# Autodesk Inventor assembly: Assembly10
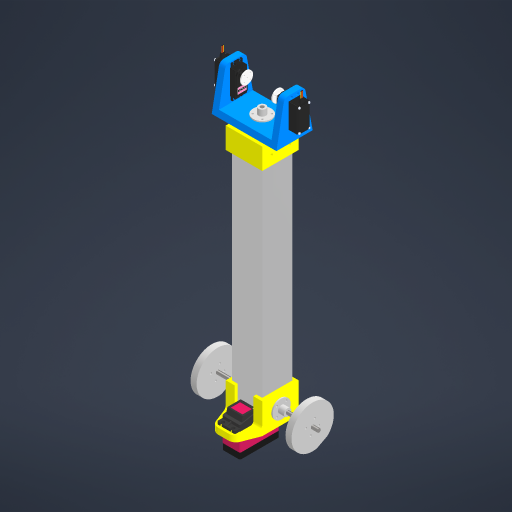
[picture p0: Inventor's stored thumbnail of the model, 512x512]
Saved by Autodesk Inventor 2023 (Build 270158000, 158)
## iProperties
Created: 2023-08-13
Part Number: Assembly10
Document SubType Name: Assembly
Designer: Abhinav
Author: Abhinav
## Documents named in this file (11)
- C:\Users\Abhinav\Desktop\GRID\ARM 3\Hand\00_Hand.iam
- C:\Users\Abhinav\Desktop\3D Library\60 kg cm Servo.ipt
- C:\Users\Abhinav\Desktop\GRID\ARM 3\Hand\Hand-Link.ipt
- C:\Users\Abhinav\Desktop\GRID\ARM 3\Hand\Servo-house.ipt
- C:\Users\Abhinav\Desktop\GRID\ARM 3\Hand\Bear-house.ipt
- C:\Users\Abhinav\Desktop\GRID\ARM 3\Hand\Flange.ipt
- C:\Users\Abhinav\Desktop\GRID\ARM 3\Hand\Shaft.ipt
- C:\Users\Abhinav\Desktop\GRID\ARM 3\Hand\Pulley-70.ipt
- C:\Users\Abhinav\Desktop\GRID\ARM 3\Hand\Hand-End Fork.ipt
- C:\Users\Abhinav\Desktop\3D Library\Servo MG964R.ipt
- C:\Users\Abhinav\Desktop\3D Library\Servo Horn.ipt
## Components (17 placed, 10 different names)
1. 60 kg cm Servo:1 — Mate:4, Mate:5, Mate:6
2. Hand-Link:1 — Mate:1, Mate:2, Mate:3, Mate:11, Mate:12, Mate:13, Mate:20, Mate:21, Flush:1, Flush:2, Mate:30, Mate:32
3. Servo-house:1 — Mate:1, Mate:2, Mate:3, Mate:4, Mate:5, Mate:6, Mate:22, Mate:23, Mate:24, Mate:25, Mate:26, Mate:27
4. Bear-house:1 — Mate:11, Mate:12, Mate:13, Mate:34, Mate:39
5. Flange:3 — Mate:22, Mate:26, Mate:27, Mate:28
6. Flange:4 — Mate:23, Mate:24, Mate:25, Mate:29
7. Shaft:1 — Flush:2, Mate:29, Mate:31
8. Shaft:2 — Flush:1, Mate:28, Mate:33
9. Pulley-70:1 — Mate:30, Mate:31, Flush:3
10. Pulley-70:2 — Mate:32, Mate:33, Flush:3
11. Hand-End Fork:1 — Mate:35, Mate:36, Mate:37, Mate:38, Mate:39, Mate:40, Mate:41, Mate:42, Mate:43, Mate:44, Mate:45
12. Shaft:3 — Mate:34, Mate:38, Flush:4
13. Flange:5 — Mate:35, Mate:36, Mate:37, Flush:4
14. Servo MG964R:1 — Mate:43, Mate:44, Mate:45, Mate:47, Mate:48
15. Servo MG964R:2 — Mate:40, Mate:41, Mate:42, Mate:46, Mate:49
16. Servo Horn:1 — Mate:46, Mate:49
17. Servo Horn:2 — Mate:47, Mate:48
## Relationships (43: Mate 39, Flush 4)
- Mate:1: Hand-Link:1 ↔ Servo-house:1
- Mate:2 (0.15 mm): Hand-Link:1 ↔ Servo-house:1
- Mate:3: Hand-Link:1 ↔ Servo-house:1
- Mate:4: 60 kg cm Servo:1 ↔ Servo-house:1
- Mate:5: 60 kg cm Servo:1 ↔ Servo-house:1
- Mate:6: 60 kg cm Servo:1 ↔ Servo-house:1
- Mate:11: Hand-Link:1 ↔ Bear-house:1
- Mate:12 (0.15 mm): Hand-Link:1 ↔ Bear-house:1
- Mate:13: Hand-Link:1 ↔ Bear-house:1
- Mate:20: Hand-Link:1
- Mate:21: Hand-Link:1
- Mate:22: Servo-house:1 ↔ Flange:3
- Mate:23: Servo-house:1 ↔ Flange:4
- Mate:24: Servo-house:1 ↔ Flange:4
- Mate:25: Servo-house:1 ↔ Flange:4
- Mate:26: Servo-house:1 ↔ Flange:3
- Mate:27: Servo-house:1 ↔ Flange:3
- Flush:1: Hand-Link:1 ↔ Shaft:2
- Mate:28: Flange:3 ↔ Shaft:2
- Flush:2: Hand-Link:1 ↔ Shaft:1
- Mate:29: Flange:4 ↔ Shaft:1
- Mate:30 (48.522 mm): Hand-Link:1 ↔ Pulley-70:1
- Mate:31: Shaft:1 ↔ Pulley-70:1
- Mate:32 (48.522 mm): Hand-Link:1 ↔ Pulley-70:2
- Mate:33: Shaft:2 ↔ Pulley-70:2
- Flush:3: Pulley-70:1 ↔ Pulley-70:2
- Mate:34: Bear-house:1 ↔ Shaft:3
- Mate:35: Hand-End Fork:1 ↔ Flange:5
- Mate:36: Hand-End Fork:1 ↔ Flange:5
- Mate:37: Hand-End Fork:1 ↔ Flange:5
- Mate:38: Hand-End Fork:1 ↔ Shaft:3
- Flush:4: Shaft:3 ↔ Flange:5
- Mate:39 (5 mm): Bear-house:1 ↔ Hand-End Fork:1
- Mate:40: Hand-End Fork:1 ↔ Servo MG964R:2
- Mate:41: Hand-End Fork:1 ↔ Servo MG964R:2
- Mate:42: Hand-End Fork:1 ↔ Servo MG964R:2
- Mate:43: Hand-End Fork:1 ↔ Servo MG964R:1
- Mate:44: Hand-End Fork:1 ↔ Servo MG964R:1
- Mate:45: Hand-End Fork:1 ↔ Servo MG964R:1
- Mate:46: Servo MG964R:2 ↔ Servo Horn:1
- Mate:47: Servo MG964R:1 ↔ Servo Horn:2
- Mate:48: Servo MG964R:1 ↔ Servo Horn:2
- Mate:49: Servo MG964R:2 ↔ Servo Horn:1
